# Autodesk Inventor assembly: Constant Spring Jig
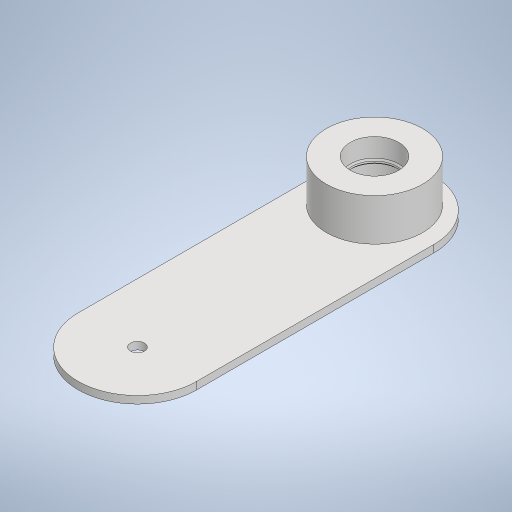
[picture p0: Inventor's stored thumbnail of the model, 512x512]
Saved by Autodesk Inventor 2023.4 (Build 274418000, 418)
## iProperties
Created: 2024-05-13
Part Number: Constant Spring Jig
Document SubType Name: Assembly
Designer: Nathan Cai
Author: Nathan Cai
## Documents named in this file (3)
- E:\Documents\Inventor\Misc\Constant Spring Jig.iam
- E:\Documents\Inventor\Misc\Base.ipt
- E:\Documents\Inventor\Misc\Spool.ipt
## Components (2 placed, 2 different names)
1. Base:1 — Mate:1, Mate:2
2. Spool:1 — Mate:1, Mate:2
## Relationships (2: Mate 2)
- Mate:1: Base:1 ↔ Spool:1
- Mate:2 (1 mm): Base:1 ↔ Spool:1
